# Autodesk Inventor assembly: legs_asm
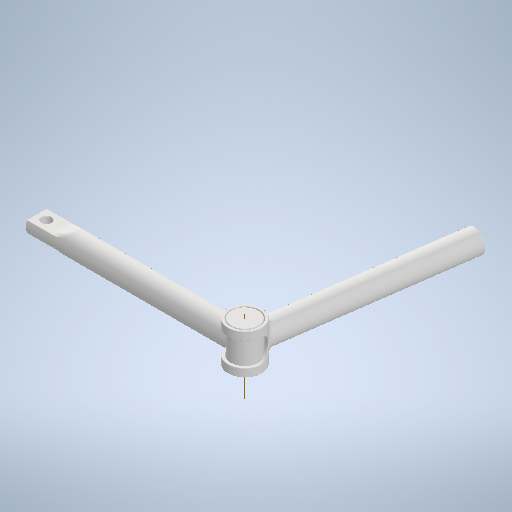
[picture p0: Inventor's stored thumbnail of the model, 512x512]
Saved by Autodesk Inventor 2025.1 (Build 291241000, 241)
## iProperties
Created: 2024-11-01
Part Number: legs_asm
Document SubType Name: Assembly
Designer: ZOMBULLI
Author: ZOMBULLI
## Documents named in this file (3)
- C:\Users\zombulli\OneDrive - Carl Zeiss AG\Desktop\DHBW\Semester 5\mte380\Stewart Platform_new\legs_asm.iam
- C:\Users\zombulli\OneDrive - Carl Zeiss AG\Desktop\DHBW\Semester 5\mte380\Stewart Platform_new\female_leg.ipt
- C:\Users\zombulli\OneDrive - Carl Zeiss AG\Desktop\DHBW\Semester 5\mte380\Stewart Platform_new\male_leg.ipt
## Components (2 placed, 2 different names)
1. female_leg:1 — Passend:1, Fluchtend:1, Winkel:1
2. male_leg:1 — Passend:1, Fluchtend:1, Winkel:1
## Relationships (3: Mate 1, Flush 1, Angle 1)
- Passend:1 [Mate]: female_leg:1 ↔ male_leg:1
- Fluchtend:1 [Flush]: female_leg:1 ↔ male_leg:1
- Winkel:1 [Angle] (82 deg): female_leg:1 ↔ male_leg:1
